# Autodesk Inventor assembly: !odom_pod
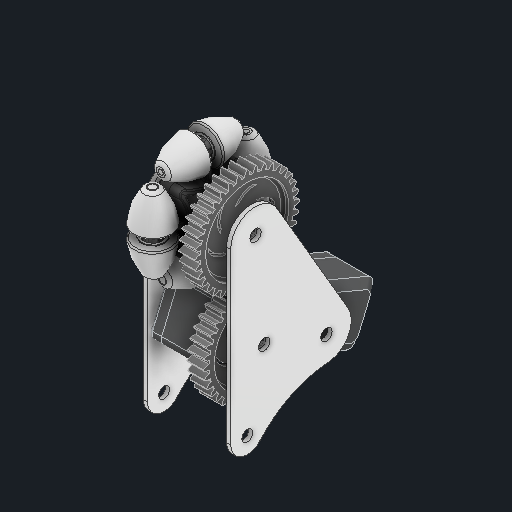
[picture p0: Inventor's stored thumbnail of the model, 512x512]
Saved by Autodesk Inventor 2024 (Build 280153000, 153)
## iProperties
Created: 2024-01-17
Part Number: !odom_pod
Document SubType Name: Assembly
Designer: avere
Author: avere
## Documents named in this file (5)
- C:\Users\avere\Documents\rbp_cad\zoomba_v0.3\chassis\odometry\!odom_pod.iam
- C:\Users\avere\Documents\rbp_cad\VEX-CAD-Inventor-1.41\Motion\Wheels\Omni Wheel\2” Omni-Directional Wheel (276-9044)\2” Omni-Directional Wheel (276-9044).ipt
- C:\Users\avere\Documents\rbp_cad\VEX-CAD-Inventor-1.41\Electronics\Sensors\V5 Rotation Sensor.ipt
- C:\Users\avere\Documents\rbp_cad\VEX-CAD-Inventor-1.41\Motion\Gears\LS 36T Gear.ipt
- C:\Users\avere\Documents\rbp_cad\zoomba_v0.3\chassis\odometry\custom_parts\pod_gusset.ipt
## Components (6 placed, 4 different names)
1. 2” Omni-Directional Wheel (276-9044):1 — Insert:2
2. V5 Rotation Sensor:1 — Insert:1, Insert:6
3. LS 36T Gear:1 — Insert:2, Insert:5
4. LS 36T Gear:2 — Insert:1, Insert:4
5. pod_gusset:1 — Insert:6
6. pod_gusset:2 — Insert:4, Insert:5
## Relationships (5: Insert 5)
- Insert:1: V5 Rotation Sensor:1 ↔ LS 36T Gear:2
- Insert:2 (2.3813 mm): 2” Omni-Directional Wheel (276-9044):1 ↔ LS 36T Gear:1
- Insert:4: LS 36T Gear:2 ↔ pod_gusset:2
- Insert:5: LS 36T Gear:1 ↔ pod_gusset:2
- Insert:6: V5 Rotation Sensor:1 ↔ pod_gusset:1
